# Autodesk Inventor assembly: support assembly
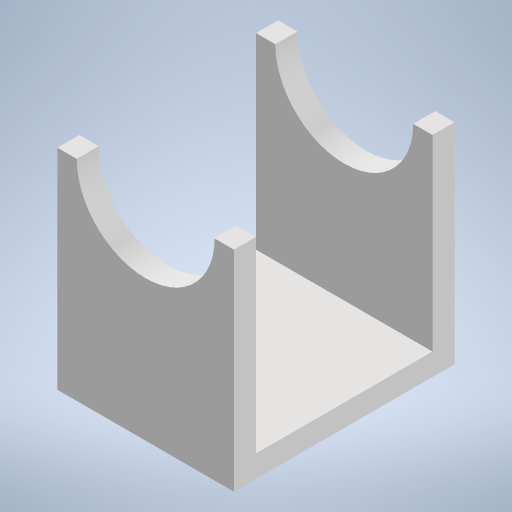
[picture p0: Inventor's stored thumbnail of the model, 512x512]
Saved by Autodesk Inventor 2023 (Build 270158000, 158)
## iProperties
Created: 2022-09-29
Part Number: support assembly
Document SubType Name: Assembly
Designer: station
Author: station
## Documents named in this file (3)
- C:\Users\station\Documents\Project\Liquid-engine-cooling-system\design files\ethanol engine 6\Aluminium engine v2\support assembly.iam
- C:\Users\station\Documents\Project\Liquid-engine-cooling-system\design files\ethanol engine 6\Aluminium engine v2\Weldedsupportpart2.ipt
- C:\Users\station\Documents\Project\Liquid-engine-cooling-system\design files\ethanol engine 6\Aluminium engine v2\Weldedsupportpart1.ipt
## Components (3 placed, 2 different names)
1. Weldedsupportpart2:1 — Mate:1, Flush:1, Flush:2, Flush:3, Mate:3
2. Weldedsupportpart1:1 — Mate:2, Flush:3, Mate:3
3. Weldedsupportpart1:2 — Mate:1, Flush:1, Flush:2, Mate:2
## Relationships (6: Mate 3, Flush 3)
- Mate:1: Weldedsupportpart2:1 ↔ Weldedsupportpart1:2
- Flush:1: Weldedsupportpart2:1 ↔ Weldedsupportpart1:2
- Flush:2: Weldedsupportpart2:1 ↔ Weldedsupportpart1:2
- Mate:2: Weldedsupportpart1:1 ↔ Weldedsupportpart1:2
- Flush:3: Weldedsupportpart2:1 ↔ Weldedsupportpart1:1
- Mate:3: Weldedsupportpart2:1 ↔ Weldedsupportpart1:1
